# Autodesk Inventor assembly: Base Chassis Assembly
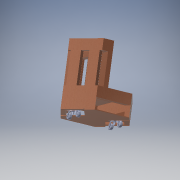
[picture p0: Inventor's stored thumbnail of the model, 180x180]
Saved by Autodesk Inventor 2017 (Build 210142000, 142)
## iProperties
Created: 2018-10-18
Part Number: Base Chassis Assembly
Document SubType Name: Assembly
Designer: Dell
Author: Dell
## Documents named in this file (12)
- C:\Users\Dell\Documents\GitHub\tr2\Base\Base Chassis Assembly.iam
- C:\Users\Dell\Documents\GitHub\tr2\BA01.ipt
- C:\Users\Dell\Documents\GitHub\tr2\BA02.ipt
- C:\Users\Dell\Documents\GitHub\tr2\Base\BA07.ipt
- C:\Users\Dell\Documents\GitHub\tr2\Base\BA11.ipt
- C:\Users\Dell\Documents\GitHub\tr2\Base\BA015.ipt
- C:\Users\Dell\Documents\GitHub\tr2\Base\Caster 2in.ipt
- C:\Users\Dell\Documents\GitHub\tr2\Base\BA16.ipt
- C:\Users\Dell\Documents\GitHub\tr2\Base\BA17.ipt
- C:\Users\Dell\Documents\GitHub\tr2\Base\BA18.ipt
- C:\Users\Dell\Documents\GitHub\tr2\Base\BA22.ipt
- C:\Users\Dell\Documents\GitHub\tr2\Base\BA23.ipt
## Components (35 placed, 11 different names)
1. BA01:1
2. BA01:2 — Flush:33, Mate:90
3. BA01:3 — Flush:41, Mate:84, Flush:51, Mate:89
4. BA01:4 — Flush:24, Flush:46, Flush:49, Flush:50
5. BA01:5 — Flush:32, Mate:65, Mate:67, Mate:88
6. BA01:6
7. BA01:7 — Mate:45, Flush:25, Mate:60, Flush:48
8. BA01:8 — Mate:47, Flush:26, Mate:49, Mate:55
9. BA01:9 — Mate:46, Mate:48, Mate:50, Mate:56
10. BA01:10 — Flush:24, Mate:45, Flush:25, Mate:61
11. BA02:2 — Mate:66, Mate:67, Flush:33
12. BA02:5 — Flush:32, Mate:65, Mate:66, Flush:53
13. BA07:4 — Mate:76, Flush:38, Flush:42, Flush:43, Mate:82, Flush:45, Flush:56, Flush:57
14. BA07:5 — Mate:69, Mate:75, Flush:37, Flush:39, Mate:78, Mate:79, Flush:40, Flush:52, Mate:92, Flush:55
15. BA11:1 — Mate:68, Flush:34, Flush:53
16. BA015:1 — Mate:46, Mate:47, Mate:48
17. BA16:1 — Flush:26, Mate:49, Mate:50, Mate:51, Mate:53, Mate:54, Flush:27, Flush:29
18. BA16:2 — Mate:60, Mate:61, Flush:29, Flush:30, Flush:31
19. BA17:1 — Mate:68, Flush:34, Mate:69, Mate:70, Flush:35, Flush:36, Mate:73, Flush:39, Flush:42, Flush:43, Flush:44, Mate:81, Flush:47, Flush:52
20. BA18:1 — Mate:70, Flush:35
21. BA18:2 — Flush:36, Mate:73, Mate:94
22. Caster 2in:1 — Mate:51, Flush:27, Mate:55, Mate:63
23. Caster 2in:2 — Mate:53, Mate:54, Mate:56, Mate:62
24. Caster 2in:3 — Flush:31, Mate:63
25. Caster 2in:4 — Mate:62, Flush:30
26. BA22:1 — Mate:75, Flush:37, Flush:47, Flush:54
27. BA22:2 — Mate:76, Flush:38, Flush:44, Mate:81, Mate:93
28. BA01:11 — Mate:78, Mate:79, Flush:40, Flush:41, Mate:80, Mate:83, Mate:91
29. BA01:12 — Mate:80, Mate:82, Flush:45, Flush:46, Mate:86, Mate:87, Mate:94
30. BA23:1 — Mate:83, Flush:48, Mate:84, Mate:85
31. BA23:2 — Mate:85, Flush:49, Mate:86
32. BA23:3 — Flush:50, Mate:87, Mate:88
33. BA23:4 — Flush:51, Mate:89, Mate:90, Mate:91
34. BA23:5 — Mate:92, Flush:54, Flush:55
35. BA23:6 — Mate:93, Flush:56, Flush:57
## Relationships (102: Mate 64, Flush 38)
- [Mate]: BA01:1 ↔ BA01:6
- [Mate]: BA01:2 ↔ BA01:6
- [Mate]: BA01:2 ↔ BA01:6
- [Mate]: BA01:2 ↔ BA01:6
- [Flush]: BA01:1 ↔ BA01:6
- [Mate]: BA01:1 ↔ BA01:6
- [Mate]: BA01:2 ↔ BA01:3
- [Mate]: BA01:2 ↔ BA01:3
- [Flush]: BA01:2 ↔ BA01:3
- [Mate]: BA01:1 ↔ BA01:5
- [Flush]: BA01:1 ↔ BA01:5
- [Mate]: BA01:1 ↔ BA01:5
- [Mate]: BA01:4 ↔ BA01:5
- [Flush]: BA01:4 ↔ BA01:5
- [Mate]: BA01:4 ↔ BA01:5
- [Mate]: BA01:3 ↔ BA01:7
- [Mate]: BA01:3 ↔ BA01:7
- [Mate]: BA01:2 ↔ BA01:7
- [Flush]: BA01:6 ↔ BA01:8
- [Mate]: BA01:2 ↔ BA01:8
- [Mate]: BA01:6 ↔ BA01:8
- [Mate]: BA01:6 ↔ BA01:8
- [Mate]: BA01:8 ↔ BA01:9
- [Mate]: BA01:5 ↔ BA01:9
- [Mate]: BA01:1 ↔ BA01:9
- [Mate] (171.45 mm): BA07:4 ↔ BA11:1
- Flush:24: BA01:4 ↔ BA01:10
- Mate:45: BA01:7 ↔ BA01:10
- Flush:25: BA01:7 ↔ BA01:10
- Mate:46: BA01:9 ↔ BA015:1
- Mate:47: BA01:8 ↔ BA015:1
- Mate:48: BA01:9 ↔ BA015:1
- Flush:26 (19.05 mm): BA01:8 ↔ BA16:1
- Mate:49: BA01:8 ↔ BA16:1
- Mate:50: BA01:9 ↔ BA16:1
- Mate:51: BA16:1 ↔ Caster 2in:1
- Mate:53: BA16:1 ↔ Caster 2in:2
- Mate:54: BA16:1 ↔ Caster 2in:2
- Flush:27: BA16:1 ↔ Caster 2in:1
- Mate:55 (12.7 mm): BA01:8 ↔ Caster 2in:1
- Mate:56 (12.7 mm): BA01:9 ↔ Caster 2in:2
- [Mate]: BA16:2 ↔ Caster 2in:3
- [Mate]: BA16:2 ↔ Caster 2in:4
- Mate:60: BA01:7 ↔ BA16:2
- Mate:61: BA01:10 ↔ BA16:2
- Flush:29: BA16:1 ↔ BA16:2
- Mate:62: Caster 2in:2 ↔ Caster 2in:4
- Flush:30: BA16:2 ↔ Caster 2in:4
- Flush:31: BA16:2 ↔ Caster 2in:3
- Mate:63: Caster 2in:1 ↔ Caster 2in:3
- Flush:32: BA01:5 ↔ BA02:5
- Mate:65: BA01:5 ↔ BA02:5
- Mate:66: BA02:2 ↔ BA02:5
- Mate:67: BA01:5 ↔ BA02:2
- Flush:33: BA01:2 ↔ BA02:2
- Mate:68: BA11:1 ↔ BA17:1
- Flush:34: BA11:1 ↔ BA17:1
- Mate:69 (38.1 mm): BA07:5 ↔ BA17:1
- Mate:70: BA17:1 ↔ BA18:1
- Flush:35: BA17:1 ↔ BA18:1
- Flush:36: BA17:1 ↔ BA18:2
- Mate:73: BA17:1 ↔ BA18:2
- Mate:75: BA07:5 ↔ BA22:1
- Flush:37 (38.1 mm): BA07:5 ↔ BA22:1
- Mate:76: BA07:4 ↔ BA22:2
- Flush:38 (38.1 mm): BA07:4 ↔ BA22:2
- Flush:39: BA07:5 ↔ BA17:1
- Mate:78: BA07:5 ↔ BA01:11
- Mate:79: BA07:5 ↔ BA01:11
- Flush:40: BA07:5 ↔ BA01:11
- Flush:41: BA01:3 ↔ BA01:11
- Mate:80: BA01:11 ↔ BA01:12
- Flush:42: BA07:4 ↔ BA17:1
- Flush:43: BA07:4 ↔ BA17:1
- Flush:44: BA17:1 ↔ BA22:2
- Mate:81: BA17:1 ↔ BA22:2
- Mate:82: BA07:4 ↔ BA01:12
- Flush:45: BA07:4 ↔ BA01:12
- Flush:46: BA01:4 ↔ BA01:12
- Flush:47: BA17:1 ↔ BA22:1
- Mate:83: BA01:11 ↔ BA23:1
- Flush:48: BA01:7 ↔ BA23:1
- Mate:84: BA01:3 ↔ BA23:1
- Mate:85: BA23:1 ↔ BA23:2
- Flush:49: BA01:4 ↔ BA23:2
- Mate:86: BA01:12 ↔ BA23:2
- Flush:50: BA01:4 ↔ BA23:3
- Mate:87: BA01:12 ↔ BA23:3
- Mate:88: BA01:5 ↔ BA23:3
- Flush:51: BA01:3 ↔ BA23:4
- Mate:89: BA01:3 ↔ BA23:4
- Mate:90: BA01:2 ↔ BA23:4
- Flush:52: BA07:5 ↔ BA17:1
- Mate:91: BA01:11 ↔ BA23:4
- Flush:53: BA02:5 ↔ BA11:1
- Mate:92: BA07:5 ↔ BA23:5
- Flush:54: BA22:1 ↔ BA23:5
- Flush:55: BA07:5 ↔ BA23:5
- Mate:93: BA22:2 ↔ BA23:6
- Flush:56: BA07:4 ↔ BA23:6
- Flush:57: BA07:4 ↔ BA23:6
- Mate:94: BA18:2 ↔ BA01:12
## Named parameters: d115_d98 = 0 mm, d122_d101 = 0 mm
